# Autodesk Inventor assembly: MotorAssembled
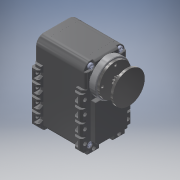
[picture p0: Inventor's stored thumbnail of the model, 180x180]
Saved by Autodesk Inventor 2019 (Build 230136000, 136)
## iProperties
Created: 2022-08-06
Part Number: MotorAssembled
Document SubType Name: Assembly
Designer: zreik
Author: zreik
## Documents named in this file (3)
- D:\Documents\HIAST\4th year\4th Year Project\Design\MotorAssembled.iam
- D:\Documents\HIAST\4th year\4th Year Project\Design\AX-12A\AX-12A.iam
- D:\Documents\HIAST\4th year\4th Year Project\Design\Pulley.ipt
## Components (2 placed, 2 different names)
1. AX-12A:1 [sub-assembly] — Flush:1, Mate:1, Flush:2, Mate:2, Mate:3, Mate:4
2. Pulley:1 — Mate:2, Mate:3, Mate:4
## Relationships (6: Mate 4, Flush 2)
- Flush:1: AX-12A:1
- Mate:1: AX-12A:1
- Flush:2: AX-12A:1
- Mate:2: AX-12A:1 ↔ Pulley:1
- Mate:3: AX-12A:1 ↔ Pulley:1
- Mate:4: AX-12A:1 ↔ Pulley:1
